# Autodesk Inventor assembly: whole project
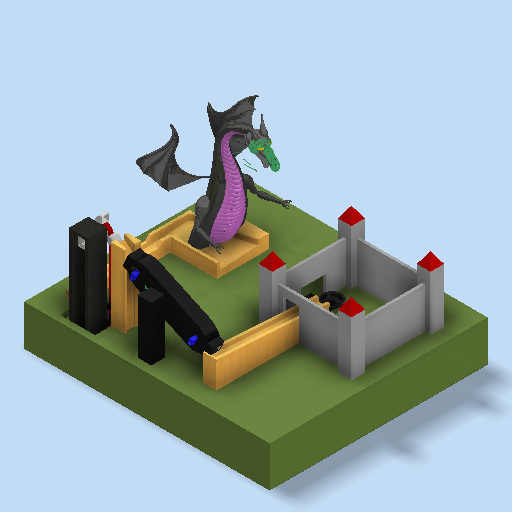
[picture p0: Inventor's stored thumbnail of the model, 512x512]
Saved by Autodesk Inventor 2025.3 (Build 293356000, 356)
## iProperties
Created: 2026-04-18
Part Number: whole project
Document SubType Name: Assembly
Designer: mosta
Author: mosta
## Documents named in this file (11)
- C:\Users\mosta\OneDrive\Documents\Inventor\Basics of mech\whole project.iam
- C:\Users\mosta\OneDrive\Documents\Inventor\Basics of mech\project's base.ipt
- C:\Users\mosta\OneDrive\Documents\Inventor\Basics of mech\sorting.iam
- C:\Users\mosta\OneDrive\Documents\Inventor\Basics of mech\sorting holder.ipt
- C:\Users\mosta\OneDrive\Documents\Inventor\Basics of mech\liftin to sorting.ipt
- C:\Users\mosta\OneDrive\Documents\Inventor\Basics of mech\Castle.ipt
- C:\Users\mosta\OneDrive\Documents\Inventor\Basics of mech\shooting FINAL.ipt
- C:\Users\mosta\OneDrive\Documents\Inventor\Basics of mech\dragon.ipt
- C:\Users\mosta\OneDrive\Documents\Inventor\Basics of mech\sorting to castle.ipt
- C:\Users\mosta\OneDrive\Documents\Inventor\Basics of mech\simplified lifting assembly.iam
- C:\Users\mosta\OneDrive\Documents\Inventor\Basics of mech\dragon to lifting.ipt
## Components (10 placed, 10 different names)
1. project's base:1 — Angle:1, Flush:1, Flush:4, Mate:14, Flush:12, Flush:20, Flush:26, Mate:26, Mate:28, Mate:30, Mate:31, Mate:32, Flush:30, Mate:35
2. sorting:1 [sub-assembly] — Flush:24, Mate:25, Flush:25, Mate:27, Flush:27, Flush:28, Flush:29
3. sorting holder:1 — Flush:24, Mate:25, Flush:25, Flush:26, Mate:26
4. Castle:1 — Mate:14, Mate:15, Flush:12, Mate:19, Flush:21, Flush:23, Mate:24
5. shooting FINAL:1 — Flush:20, Mate:19, Mate:20, Mate:27
6. dragon:1 — Flush:23, Mate:24, Mate:34
7. sorting to castle:1 — Flush:27, Mate:28, Flush:28
8. simplified lifting assembly:1 [sub-assembly] — Mate:30, Mate:31, Flush:29, Mate:33
9. dragon to lifting:1 — Mate:32, Flush:30, Mate:33, Mate:34
10. liftin to sorting:1 — Mate:35
## Relationships (29: Mate 15, Flush 13, Angle 1)
- Angle:1 (0 deg): project's base:1
- Flush:1: project's base:1
- Flush:4: project's base:1
- Mate:14: project's base:1 ↔ Castle:1
- Mate:15 (80 mm): Castle:1
- Flush:12 (130 mm): project's base:1 ↔ Castle:1
- Flush:20 (20 mm): project's base:1 ↔ shooting FINAL:1
- Mate:19: Castle:1 ↔ shooting FINAL:1
- Flush:21: Castle:1
- Mate:20 (-20 mm): shooting FINAL:1
- Flush:23: Castle:1 ↔ dragon:1
- Mate:24 (350 mm): Castle:1 ↔ dragon:1
- Flush:24: sorting:1 ↔ sorting holder:1
- Mate:25: sorting:1 ↔ sorting holder:1
- Flush:25: sorting:1 ↔ sorting holder:1
- Flush:26 (30 mm): project's base:1 ↔ sorting holder:1
- Mate:26: project's base:1 ↔ sorting holder:1
- Mate:27: sorting:1 ↔ shooting FINAL:1
- Flush:27: sorting:1 ↔ sorting to castle:1
- Mate:28: project's base:1 ↔ sorting to castle:1
- Flush:28 (-10 mm): sorting:1 ↔ sorting to castle:1
- Mate:30: project's base:1 ↔ simplified lifting assembly:1
- Mate:31: project's base:1 ↔ simplified lifting assembly:1
- Flush:29 (-20 mm): sorting:1 ↔ simplified lifting assembly:1
- Mate:32: project's base:1 ↔ dragon to lifting:1
- Flush:30 (-60 mm): project's base:1 ↔ dragon to lifting:1
- Mate:33: simplified lifting assembly:1 ↔ dragon to lifting:1
- Mate:34: dragon:1 ↔ dragon to lifting:1
- Mate:35: project's base:1 ↔ liftin to sorting:1
